# Autodesk Inventor assembly: клешня сбока
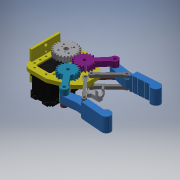
[picture p0: Inventor's stored thumbnail of the model, 180x180]
Saved by Autodesk Inventor 2019 (Build 230136000, 136)
## iProperties
Created: 2019-08-18
Part Number: клешня сбока
Material: Типовые
Document SubType Name: Assembly
Designer: Петров Иван
Mass: 102.999 g
Surface Area: 462.88 cm^2
Volume: 97.4501 cm^3
Density: 1.05694 g/cm^3
Author: Петров Иван
## Documents named in this file (10)
- E:\IVAN\Kvantoriada2019\optimal_gripper\hardware\КВ33.044.200 - Сборка зажима.iam
- E:\IVAN\Kvantoriada2019\optimal_gripper\hardware\КВ33.044.201 - Опора зажимного механизма.ipt
- E:\IVAN\Kvantoriada2019\optimal_gripper\hardware\КВ33.044.202 -Прихват.ipt
- E:\IVAN\Kvantoriada2019\optimal_gripper\hardware\КВ33.044.205 - Рычаг приводной 17 зубьев.ipt
- E:\IVAN\Kvantoriada2019\optimal_gripper\hardware\КВ33.044.206 - Рычаг приводной 16 зубьев.ipt
- E:\IVAN\Kvantoriada2019\optimal_gripper\hardware\КВ33.044.204 -Рычаг тонкий.ipt
- E:\IVAN\Kvantoriada2019\optimal_gripper\hardware\КВ33.044.203 - Рычаг толстый.ipt
- E:\IVAN\Kvantoriada2019\optimal_gripper\hardware\Стандартные изделия\Сервомотор Dynamixel AX-12A\AX-12.iam
- E:\IVAN\Kvantoriada2019\optimal_gripper\hardware\КВ33.044.102 - Колесо зубчатое сервомотора.ipt
- E:\IVAN\Kvantoriada2019\optimal_gripper\hardware\КВ33.044.207 - Крепление вакумной присоски.ipt
## Components (14 placed, 9 different names)
1. КВ33.044.201 - Опора зажимного механизма:1 — Совмещение:11, Совмещение:14, Совмещение:17, Совмещение:18, Совмещение:19, Совмещение:21, Совмещение:23, Совмещение:24, Совмещение:25, Совмещение:34, Совмещение:35, Совмещение:37, Совмещение:38, Совмещение:40, Совмещение:41, Совмещение:42, Заподлицо:2, Совмещение:46
2. КВ33.044.202 -Прихват:1 — Совмещение:12, Совмещение:13, Совмещение:15, Совмещение:16, Совмещение:26, Совмещение:33, Совмещение:36
3. КВ33.044.202 -Прихват:2 — Совмещение:9, Совмещение:10, Совмещение:20, Совмещение:22, Совмещение:32, Совмещение:39
4. КВ33.044.204 -Рычаг тонкий:1 — Совмещение:9, Совмещение:10, Совмещение:11, Совмещение:45
5. КВ33.044.204 -Рычаг тонкий:2 — Совмещение:12, Совмещение:13, Совмещение:14
6. КВ33.044.204 -Рычаг тонкий:3 — Совмещение:15, Совмещение:16, Совмещение:17
7. КВ33.044.204 -Рычаг тонкий:4 — Совмещение:18, Совмещение:19, Совмещение:20
8. КВ33.044.203 - Рычаг толстый:1 — Совмещение:24, Совмещение:25, Совмещение:26, Совмещение:33
9. КВ33.044.203 - Рычаг толстый:2 — Совмещение:21, Совмещение:22, Совмещение:23, Совмещение:32
10. AX-12:1 [sub-assembly] — Совмещение:40, Совмещение:41, Совмещение:42, Совмещение:43, Совмещение:44
11. КВ33.044.102 - Колесо зубчатое сервомотора:1 — Направление навивки:1, Совмещение:43, Совмещение:44
12. КВ33.044.205 - Рычаг приводной 17 зубьев:1 — Совмещение:34, Совмещение:35, Совмещение:36, Направление навивки:1, Направление навивки:2
13. КВ33.044.206 - Рычаг приводной 16 зубьев:1 — Совмещение:37, Совмещение:38, Совмещение:39, Направление навивки:2
14. КВ33.044.207 - Крепление вакумной присоски:1 — Заподлицо:2, Совмещение:45, Совмещение:46
## Relationships (36: Mate 33, RelateRotation 2, Flush 1)
- Совмещение:9 [Mate]: КВ33.044.202 -Прихват:2 ↔ КВ33.044.204 -Рычаг тонкий:1
- Совмещение:10 [Mate]: КВ33.044.202 -Прихват:2 ↔ КВ33.044.204 -Рычаг тонкий:1
- Совмещение:11 [Mate]: КВ33.044.201 - Опора зажимного механизма:1 ↔ КВ33.044.204 -Рычаг тонкий:1
- Совмещение:12 [Mate]: КВ33.044.202 -Прихват:1 ↔ КВ33.044.204 -Рычаг тонкий:2
- Совмещение:13 [Mate]: КВ33.044.202 -Прихват:1 ↔ КВ33.044.204 -Рычаг тонкий:2
- Совмещение:14 [Mate]: КВ33.044.201 - Опора зажимного механизма:1 ↔ КВ33.044.204 -Рычаг тонкий:2
- Совмещение:15 [Mate]: КВ33.044.202 -Прихват:1 ↔ КВ33.044.204 -Рычаг тонкий:3
- Совмещение:16 [Mate]: КВ33.044.202 -Прихват:1 ↔ КВ33.044.204 -Рычаг тонкий:3
- Совмещение:17 [Mate]: КВ33.044.201 - Опора зажимного механизма:1 ↔ КВ33.044.204 -Рычаг тонкий:3
- Совмещение:18 [Mate]: КВ33.044.201 - Опора зажимного механизма:1 ↔ КВ33.044.204 -Рычаг тонкий:4
- Совмещение:19 [Mate]: КВ33.044.201 - Опора зажимного механизма:1 ↔ КВ33.044.204 -Рычаг тонкий:4
- Совмещение:20 [Mate]: КВ33.044.202 -Прихват:2 ↔ КВ33.044.204 -Рычаг тонкий:4
- Совмещение:21 [Mate]: КВ33.044.201 - Опора зажимного механизма:1 ↔ КВ33.044.203 - Рычаг толстый:2
- Совмещение:22 [Mate]: КВ33.044.202 -Прихват:2 ↔ КВ33.044.203 - Рычаг толстый:2
- Совмещение:23 [Mate]: КВ33.044.201 - Опора зажимного механизма:1 ↔ КВ33.044.203 - Рычаг толстый:2
- Совмещение:24 [Mate]: КВ33.044.201 - Опора зажимного механизма:1 ↔ КВ33.044.203 - Рычаг толстый:1
- Совмещение:25 [Mate]: КВ33.044.201 - Опора зажимного механизма:1 ↔ КВ33.044.203 - Рычаг толстый:1
- Совмещение:26 [Mate]: КВ33.044.202 -Прихват:1 ↔ КВ33.044.203 - Рычаг толстый:1
- Совмещение:32 [Mate]: КВ33.044.202 -Прихват:2 ↔ КВ33.044.203 - Рычаг толстый:2
- Совмещение:33 [Mate]: КВ33.044.202 -Прихват:1 ↔ КВ33.044.203 - Рычаг толстый:1
- Совмещение:34 [Mate]: КВ33.044.201 - Опора зажимного механизма:1 ↔ КВ33.044.205 - Рычаг приводной 17 зубьев:1
- Совмещение:35 [Mate]: КВ33.044.201 - Опора зажимного механизма:1 ↔ КВ33.044.205 - Рычаг приводной 17 зубьев:1
- Совмещение:36 [Mate]: КВ33.044.202 -Прихват:1 ↔ КВ33.044.205 - Рычаг приводной 17 зубьев:1
- Совмещение:37 [Mate]: КВ33.044.201 - Опора зажимного механизма:1 ↔ КВ33.044.206 - Рычаг приводной 16 зубьев:1
- Совмещение:38 [Mate]: КВ33.044.201 - Опора зажимного механизма:1 ↔ КВ33.044.206 - Рычаг приводной 16 зубьев:1
- Совмещение:39 [Mate]: КВ33.044.202 -Прихват:2 ↔ КВ33.044.206 - Рычаг приводной 16 зубьев:1
- Направление навивки:1 [RelateRotation] (1.5 ul): КВ33.044.102 - Колесо зубчатое сервомотора:1 ↔ КВ33.044.205 - Рычаг приводной 17 зубьев:1
- Направление навивки:2 [RelateRotation] (1 ul): КВ33.044.205 - Рычаг приводной 17 зубьев:1 ↔ КВ33.044.206 - Рычаг приводной 16 зубьев:1
- Совмещение:40 [Mate]: КВ33.044.201 - Опора зажимного механизма:1 ↔ AX-12:1
- Совмещение:41 [Mate]: КВ33.044.201 - Опора зажимного механизма:1 ↔ AX-12:1
- Совмещение:42 [Mate]: КВ33.044.201 - Опора зажимного механизма:1 ↔ AX-12:1
- Совмещение:43 [Mate]: AX-12:1 ↔ КВ33.044.102 - Колесо зубчатое сервомотора:1
- Совмещение:44 [Mate]: AX-12:1 ↔ КВ33.044.102 - Колесо зубчатое сервомотора:1
- Заподлицо:2 [Flush] (23.625 mm): КВ33.044.201 - Опора зажимного механизма:1 ↔ КВ33.044.207 - Крепление вакумной присоски:1
- Совмещение:45 [Mate]: КВ33.044.204 -Рычаг тонкий:1 ↔ КВ33.044.207 - Крепление вакумной присоски:1
- Совмещение:46 [Mate] (-6.474 mm): КВ33.044.201 - Опора зажимного механизма:1 ↔ КВ33.044.207 - Крепление вакумной присоски:1
